# Autodesk Inventor assembly: Arms
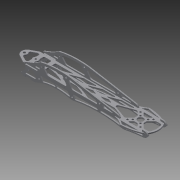
[picture p0: Inventor's stored thumbnail of the model, 180x180]
Saved by Autodesk Inventor 2014 SP1 (Build 180222100, 222)
## iProperties
Created: 2014-07-29
Part Number: Arms
Document SubType Name: Assembly
Designer: Ryan
Author: Ryan
## Documents named in this file (3)
- C:\Users\Ryan\Documents\Inventor\Quadrocopter\Frame_V1\V1\Arms.iam
- C:\Users\Ryan\Documents\Inventor\Quadrocopter\Frame_V1\V1\Arm.ipt
- C:\Users\Ryan\Documents\Inventor\Quadrocopter\Frame_V1\V1\Arm_Side.ipt
## Components (3 placed, 2 different names)
1. Arm:1 — Mate:1, Mate:2, Flush:1, Mate:3, Mate:4, Flush:2
2. Arm_Side:1 — Mate:3, Mate:4, Flush:2
3. Arm_Side:2 — Mate:1, Mate:2, Flush:1
## Relationships (6: Mate 4, Flush 2)
- Mate:1: Arm:1 ↔ Arm_Side:2
- Mate:2: Arm:1 ↔ Arm_Side:2
- Flush:1: Arm:1 ↔ Arm_Side:2
- Mate:3: Arm:1 ↔ Arm_Side:1
- Mate:4: Arm:1 ↔ Arm_Side:1
- Flush:2: Arm:1 ↔ Arm_Side:1
